# Autodesk Inventor assembly: Assembly_Cube_Openflexure_Stage_v2
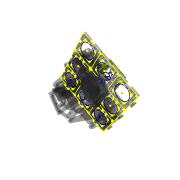
[picture p0: Inventor's stored thumbnail of the model, 180x180]
Saved by Autodesk Inventor 2019.4 (Build 234330000, 330)
## iProperties
Created: 2019-08-12
Part Number: Assembly_Cube_Openflexure_Stage_v2
Document SubType Name: Assembly
Designer: diederichbenedict
Author: diederichbenedict
## Documents named in this file (5)
- C:\Users\diederichbenedict\Dropbox\Dokumente\Promotion\PROJECTS\UC2\02_CAD\INVENTOR\uc2_v3\Assembly_Cube_Openflexure_Stage_v3.iam
- C:\Users\diederichbenedict\Dropbox\Dokumente\Promotion\PROJECTS\UC2\02_CAD\INVENTOR\uc2_v3\20_Cube_Insert_Openflexure_Deltastage_Adapter_v3.ipt
- C:\Users\diederichbenedict\Dropbox\Dokumente\Promotion\PROJECTS\UC2\02_CAD\INVENTOR\uc2_v3\00_openflexure_deltastage.ipt
- C:\Users\diederichbenedict\Dropbox\Dokumente\Promotion\PROJECTS\UC2\02_CAD\INVENTOR\uc2_v3\Assembly_Cube_empty_IM_v3.iam
- C:\Users\diederichbenedict\Dropbox\Dokumente\Promotion\PROJECTS\UC2\02_CAD\INVENTOR\uc2_v3\10_Base_puzzle_v3.ipt
## Components (12 placed, 4 different names)
1. 20_Cube_Insert_Openflexure_Deltastage_Adapter_v3:1 — Flush:2
2. 00_openflexure_deltastage:1 — Flush:2, Mate:1, Angle:1, Mate:2
3. Assembly_Cube_empty_IM_v3:3 [sub-assembly] — Angle:2, Insert:1
4. 10_Base_puzzle_v3:5 — Mate:1, Angle:1, Mate:2, Insert:1
5. 10_Base_puzzle_v3:6 — Angle:2
6. 10_Base_puzzle_v3:7
7. 10_Base_puzzle_v3:8
8. 10_Base_puzzle_v3:9
9. 10_Base_puzzle_v3:10
10. 10_Base_puzzle_v3:11
11. 10_Base_puzzle_v3:12
12. 10_Base_puzzle_v3:13
## Component patterns: (9 elements, first: 10_Base_puzzle_v3:5)
## Relationships (6: Mate 2, Angle 2, Flush 1, Insert 1)
- Flush:2: 20_Cube_Insert_Openflexure_Deltastage_Adapter_v3:1 ↔ 00_openflexure_deltastage:1
- Mate:1: 00_openflexure_deltastage:1 ↔ 10_Base_puzzle_v3:5
- Angle:1 (0 deg): 00_openflexure_deltastage:1 ↔ 10_Base_puzzle_v3:5
- Mate:2 (6 mm): 00_openflexure_deltastage:1 ↔ 10_Base_puzzle_v3:5
- Angle:2 (0 deg): Assembly_Cube_empty_IM_v3:3 ↔ 10_Base_puzzle_v3:6
- Insert:1: Assembly_Cube_empty_IM_v3:3 ↔ 10_Base_puzzle_v3:5
